# Autodesk Inventor assembly: 10.5 in Spacer
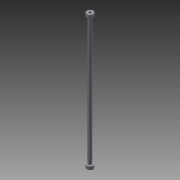
[picture p0: Inventor's stored thumbnail of the model, 180x180]
Saved by Autodesk Inventor 2015 (Build 190159000, 159)
## iProperties
Created: 2016-09-22
Part Number: 10.5 in Spacer
Document SubType Name: Assembly
Designer: L
Author: L
## Documents named in this file (5)
- C:\Users\L\Google Drive\StarStuckProject\Starstruck\Prototypes\10.5 in Spacer.iam
- 11.5 in Spacer.iam
- C:\Users\L\Google Drive\StarStuckProject\Starstruck\Imported Components\White Spacer .250in\White Spacer .250in.ipt
- C:\Users\L\Google Drive\StarStuckProject\Starstruck\Imported Components\5.00In Standoff\5.00In Standoff.ipt
- C:\Users\L\Google Drive\StarStuckProject\Starstruck\Imported Components\1.00In Coupler\1.00In Coupler.ipt
## Components (5 placed, 3 different names)
1. White Spacer .250in:1 — Mate:4, Tangent:3
2. White Spacer .250in:2 — Mate:3, Tangent:4
3. 5.00In Standoff:1 — Tangent:1, Mate:1, Flush:1, Mate:3, Tangent:4
4. 5.00In Standoff:2 — Mate:2, Tangent:2, Flush:1, Mate:4, Tangent:3
5. 1.00In Coupler:1 — Tangent:1, Mate:1, Mate:2, Tangent:2
## Relationships (9: Tangent 4, Mate 4, Flush 1)
- Tangent:1: 5.00In Standoff:1 ↔ 1.00In Coupler:1
- Mate:1: 5.00In Standoff:1 ↔ 1.00In Coupler:1
- Mate:2: 5.00In Standoff:2 ↔ 1.00In Coupler:1
- Tangent:2: 5.00In Standoff:2 ↔ 1.00In Coupler:1
- Flush:1: 5.00In Standoff:1 ↔ 5.00In Standoff:2
- Mate:3: White Spacer .250in:2 ↔ 5.00In Standoff:1
- Mate:4: White Spacer .250in:1 ↔ 5.00In Standoff:2
- Tangent:3: White Spacer .250in:1 ↔ 5.00In Standoff:2
- Tangent:4: White Spacer .250in:2 ↔ 5.00In Standoff:1
